# Autodesk Inventor assembly: 110033226_iam_05_騎樓梁架
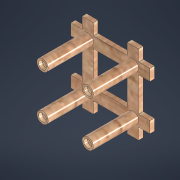
[picture p0: Inventor's stored thumbnail of the model, 180x180]
Saved by Autodesk Inventor 2022 (Build 260153000, 153)
## iProperties
Created: 2022-06-24
Part Number: 110033226_iam_05_騎樓梁架
Document SubType Name: Assembly
Designer: User
Author: User
## Documents named in this file (3)
- D:\D-disk\pomelo\大一\下學期\機械設計製圖\1100332260_LEGOproj_沒有公主城堡\110033226_iam_05_騎樓梁架.iam
- D:\D-disk\pomelo\大一\下學期\機械設計製圖\1100332260_LEGOproj_沒有公主城堡\110033226_ipt_27_騎樓梁架頂.ipt
- D:\D-disk\pomelo\大一\下學期\機械設計製圖\1100332260_LEGOproj_沒有公主城堡\110033226_ipt_26_騎樓梁架.ipt
## Components (2 placed, 2 different names)
1. 110033226_ipt_27_騎樓梁架頂:1 — 貼合:1, 貼合:2, 貼合:3
2. 110033226_ipt_26_騎樓梁架:1 — 貼合:1, 貼合:2, 貼合:3
## Relationships (3: Mate 3)
- 貼合:1 [Mate]: 110033226_ipt_27_騎樓梁架頂:1 ↔ 110033226_ipt_26_騎樓梁架:1
- 貼合:2 [Mate]: 110033226_ipt_27_騎樓梁架頂:1 ↔ 110033226_ipt_26_騎樓梁架:1
- 貼合:3 [Mate]: 110033226_ipt_27_騎樓梁架頂:1 ↔ 110033226_ipt_26_騎樓梁架:1
